# Autodesk Inventor assembly: S4x1
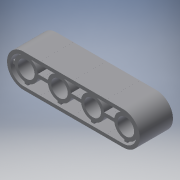
[picture p0: Inventor's stored thumbnail of the model, 180x180]
Saved by Autodesk Inventor 2019.3 (Build 233278000, 278)
## iProperties
Created: 2019-01-31
Part Number: S4x1
Document SubType Name: Assembly
Designer: Varga Daniel
Author: Varga Daniel
## Documents named in this file (4)
- C:\!_Dani\!_cloud\OneDrive\!_munka\Revolution\RevvyDemoKit\Structural parts\Beams\Straight Beams\S2+x1\S4x1.iam
- C:\!_Dani\!_cloud\OneDrive\!_munka\Revolution\RevvyDemoKit\Structural parts\Beams\beam_single_end_part.ipt
- C:\!_Dani\!_cloud\OneDrive\!_munka\Revolution\RevvyDemoKit\Structural parts\Beams\beam_single_inner_part.ipt
- C:\!_Dani\!_cloud\OneDrive\!_munka\Revolution\RevvyDemoKit\Structural parts\Beams\Straight Beams\S2+x1.iam
## Components (4 placed, 2 different names)
1. beam_single_end_part:1 — Flush:1, Flush:2, Mate:1, Flush:3, Flush:4, Mate:2
2. beam_single_end_part:2 — Flush:1, Flush:2, Mate:1
3. beam_single_inner_part:1 — Flush:3, Flush:4, Mate:2
4. beam_single_inner_part:2
## Component patterns: (2 elements, first: beam_single_inner_part:1)
## Relationships (6: Flush 4, Mate 2)
- Flush:1: beam_single_end_part:1 ↔ beam_single_end_part:2
- Flush:2: beam_single_end_part:1 ↔ beam_single_end_part:2
- Mate:1 (20 mm): beam_single_end_part:1 ↔ beam_single_end_part:2
- Flush:3: beam_single_end_part:1 ↔ beam_single_inner_part:1
- Flush:4: beam_single_end_part:1 ↔ beam_single_inner_part:1
- Mate:2: beam_single_end_part:1 ↔ beam_single_inner_part:1
